# Autodesk Inventor assembly: 5to1GearCreation_Trial_1
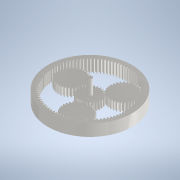
[picture p0: Inventor's stored thumbnail of the model, 180x180]
Saved by Autodesk Inventor 2022 (Build 260153000, 153)
## iProperties
Created: 2022-04-22
Part Number: 5to1GearCreation_Trial_1
Document SubType Name: Assembly
Designer: Mlees
Author: Mlees
## Documents named in this file (4)
- C:\Users\Mlees\Desktop\504Engineering\Project_0000\Designs\Design_2\Created_Parts\Gear_Folder\5to1GearCreation_Trial_1.iam
- C:\Users\Mlees\Desktop\504Engineering\Project_0000\Designs\Design_2\Created_Parts\Gear_Folder\5to1GearCreation_Trial_1\Design Accelerator\Spur Gears9.iam
- C:\Users\Mlees\Desktop\504Engineering\Project_0000\Designs\Design_2\Created_Parts\Gear_Folder\5to1GearCreation_Trial_1\Design Accelerator\Spur Gear13.ipt
- C:\Users\Mlees\Desktop\504Engineering\Project_0000\Designs\Design_2\Created_Parts\Gear_Folder\5to1GearCreation_Trial_1\Design Accelerator\Spur Gear23.ipt
## Components (5 placed, 3 different names)
1. Spur Gears:6 [sub-assembly] — Flush:4, Mate:1
2. Spur Gear1:1 — Flush:1, Flush:2, Flush:4, Mate:1, Rotation:1
3. Spur Gear2:1 — Flush:3, Rotation:1
4. Spur Gear2:2 — Flush:2, Flush:3
5. Spur Gear2:3 — Flush:1
## Relationships (6: Flush 4, Mate 1, RelateRotation 1)
- Flush:1: Spur Gear1:1 ↔ Spur Gear2:3
- Flush:2: Spur Gear1:1 ↔ Spur Gear2:2
- Flush:3: Spur Gear2:1 ↔ Spur Gear2:2
- Flush:4: Spur Gears:6 ↔ Spur Gear1:1
- Mate:1: Spur Gears:6 ↔ Spur Gear1:1
- Rotation:1 [RelateRotation] (1.447 ul): Spur Gear1:1 ↔ Spur Gear2:1
